# Autodesk Inventor assembly: Black Box
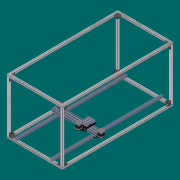
[picture p0: Inventor's stored thumbnail of the model, 180x180]
Saved by Autodesk Inventor 2016 (Build 200138000, 138)
## iProperties
Created: 2015-06-04
Part Number: Black Box
Document SubType Name: Assembly
Designer: Sawaiz Syed
Author: Sawaiz Syed
## Documents named in this file (7)
- C:\Users\Sawaiz\Documents\data\projects\cncBlackBox\blackBox.iam
- C:\Users\Sawaiz\Documents\data\projects\cncBlackBox\frame\frame.iam
- C:\Users\Sawaiz\Documents\data\projects\cncBlackBox\yAxis\yAxis.iam
- C:\Users\Sawaiz\Documents\data\projects\cncBlackBox\xAxis\xAxis.iam
- C:\Users\Sawaiz\Documents\data\projects\cncBlackBox\yAxis\ySlider.iam
- C:\Users\Sawaiz\Documents\data\projects\cncBlackBox\panels\panelA.iam
- C:\Users\Sawaiz\Documents\data\projects\cncBlackBox\panels\panelB.iam
## Components (10 placed, 6 different names)
1. frame:1 [sub-assembly] — Flush:2, Mate:2, Flush:3, Mate:4, Mate:5, Mate:6, Mate:7, Flush:5, Flush:6, Flush:7, Flush:8, Flush:9, Mate:11, Mate:12
2. yAxis:1 [sub-assembly] — Flush:1, Mate:1, Mate:3, Flush:4
3. xAxis:1 [sub-assembly] — Flush:1, Mate:1, Flush:2, Mate:2, Flush:3
4. ySlider:1 [sub-assembly] — Mate:3, Flush:4
5. panelA:1 [sub-assembly] — Mate:6, Flush:8, Mate:9, Mate:10, Mate:15
6. panelA:2 [sub-assembly] — Mate:4, Flush:7, Mate:8, Mate:9, Mate:14, Mate:16
7. panelA:3 [sub-assembly] — Mate:5, Flush:9, Mate:10
8. panelA:4 [sub-assembly] — Mate:7, Flush:5, Flush:6, Mate:8, Mate:13
9. panelB:1 [sub-assembly] — Mate:11, Mate:15, Mate:16
10. panelB:2 [sub-assembly] — Mate:12, Mate:13, Mate:14
## Relationships (25: Mate 16, Flush 9)
- Flush:1 (-62.95 mm): yAxis:1 ↔ xAxis:1
- Mate:1 (0.85 mm): yAxis:1 ↔ xAxis:1
- Flush:2: frame:1 ↔ xAxis:1
- Mate:2: frame:1 ↔ xAxis:1
- Flush:3 (90 mm): frame:1 ↔ xAxis:1
- Mate:3 (0.85 mm): yAxis:1 ↔ ySlider:1
- Flush:4 (-52.95 mm): yAxis:1 ↔ ySlider:1
- Mate:4: frame:1 ↔ panelA:2
- Mate:5: frame:1 ↔ panelA:3
- Mate:6: frame:1 ↔ panelA:1
- Mate:7: frame:1 ↔ panelA:4
- Flush:5: frame:1 ↔ panelA:4
- Flush:6: frame:1 ↔ panelA:4
- Flush:7: frame:1 ↔ panelA:2
- Mate:8: panelA:2 ↔ panelA:4
- Flush:8: frame:1 ↔ panelA:1
- Mate:9: panelA:1 ↔ panelA:2
- Flush:9: frame:1 ↔ panelA:3
- Mate:10: panelA:1 ↔ panelA:3
- Mate:11: frame:1 ↔ panelB:1
- Mate:12: frame:1 ↔ panelB:2
- Mate:13: panelA:4 ↔ panelB:2
- Mate:14: panelA:2 ↔ panelB:2
- Mate:15: panelA:1 ↔ panelB:1
- Mate:16: panelA:2 ↔ panelB:1
